# Autodesk Inventor assembly: Protochip
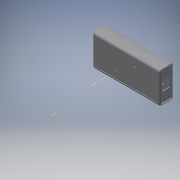
[picture p0: Inventor's stored thumbnail of the model, 180x180]
Saved by Autodesk Inventor 2016 (Build 200138000, 138)
## iProperties
Created: 2011-06-17
Part Number: Protochip
Document SubType Name: Assembly
Designer: David
Sending System: Autodesk Inventor 2011
Preprocessor: Autodesk Inventor 2011
Title: E:\Eng\Customer Service\Drawings\1593\STEP\1593Y\1593Y Assembly.stp
Author: lwalsh
## Documents named in this file (10)
- C:\Users\David\Documents\GitHub\protochip\casing\Protochip.iam
- C:\Users\David\Documents\GitHub\protochip\casing\1593Y Bottom.ipt
- C:\Users\David\Documents\GitHub\protochip\casing\1593Y Top.ipt
- C:\Users\David\Documents\GitHub\protochip\casing\1593Y Battery Cover.ipt
- C:\Users\David\Documents\GitHub\protochip\casing\1593Y Endplate.ipt
- C:\Users\David\Documents\GitHub\protochip\casing\Cheapstat.ipt
- C:\Users\David\Documents\GitHub\protochip\casing\Protochip\Design Accelerator\Bolted Connection2.iam
- C:\Users\David\Documents\GitHub\protochip\casing\Protochip\Design Accelerator\Bolted Connection3.iam
- C:\Users\David\Documents\GitHub\protochip\casing\Protochip\Design Accelerator\Bolted Connection4.iam
- C:\Users\David\Documents\GitHub\protochip\casing\Protochip\Design Accelerator\Bolted Connection5.iam
## Components (9 placed, 6 different names)
1. 1593Y Bottom:1 — Rigid:1, Slider:1, Rigid:2
2. 1593Y Top:1 — Rigid:1, Mate:1, Angle:1, Mate:4, Mate:7, Mate:9, Mate:10, Mate:14, Mate:16, Mate:18, Mate:20, Mate:22
3. 1593Y Battery Cover:1 — Slider:1
4. 1593Y Endplate:1 — Rigid:2
5. Cheapstat:1 — Mate:1, Angle:1, Mate:8, Mate:11, Mate:15, Mate:17, Mate:19, Mate:21
6. Bolted Connection:1 [sub-assembly] — Mate:15, Mate:16
7. Bolted Connection:2 [sub-assembly] — Mate:17, Mate:18
8. Bolted Connection:3 [sub-assembly] — Mate:19, Mate:20
9. Bolted Connection:4 [sub-assembly] — Mate:21, Mate:22
## Relationships (22: Mate 18, WeldJoint 2, TranslationJoint 1, Angle 1)
- Rigid:1 [WeldJoint] (0.2 mm): 1593Y Bottom:1 ↔ 1593Y Top:1
- Slider:1 [TranslationJoint]: 1593Y Bottom:1 ↔ 1593Y Battery Cover:1
- Rigid:2 [WeldJoint]: 1593Y Bottom:1 ↔ 1593Y Endplate:1
- Mate:1: 1593Y Top:1 ↔ Cheapstat:1
- Angle:1 (0 deg): 1593Y Top:1 ↔ Cheapstat:1
- Mate:4: 1593Y Top:1
- Mate:6
- Mate:7: 1593Y Top:1
- Mate:8: Cheapstat:1
- Mate:9: 1593Y Top:1
- Mate:10: 1593Y Top:1
- Mate:11: Cheapstat:1
- Mate:12
- Mate:14: 1593Y Top:1
- Mate:15: Cheapstat:1 ↔ Bolted Connection:1
- Mate:16: 1593Y Top:1 ↔ Bolted Connection:1
- Mate:17: Cheapstat:1 ↔ Bolted Connection:2
- Mate:18: 1593Y Top:1 ↔ Bolted Connection:2
- Mate:19: Cheapstat:1 ↔ Bolted Connection:3
- Mate:20: 1593Y Top:1 ↔ Bolted Connection:3
- Mate:21: Cheapstat:1 ↔ Bolted Connection:4
- Mate:22: 1593Y Top:1 ↔ Bolted Connection:4
